# Autodesk Inventor assembly: Ensamblaje
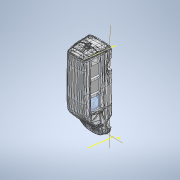
[picture p0: Inventor's stored thumbnail of the model, 180x180]
Saved by Autodesk Inventor 2021 (Build 250183000, 183)
## iProperties
Created: 2021-06-04
Part Number: Ensamblaje
Document SubType Name: Assembly
Designer: Mecatronica
Author: Mecatronica
## Documents named in this file (3)
- G:\Unidades compartidas\Robótica\Proyecto\Ensamblaje.iam
- G:\Unidades compartidas\Robótica\Proyecto\Ventanas.ipt
- G:\Unidades compartidas\Robótica\Proyecto\Carro5.ipt
## Components (2 placed, 2 different names)
1. Carro5:1 — Coincidencia:1
2. Ventanas:1 — Coincidencia:1
## Relationships (1: Mate 1)
- Coincidencia:1 [Mate]: Carro5:1 ↔ Ventanas:1
